# Autodesk Inventor assembly: Transmission Pulley
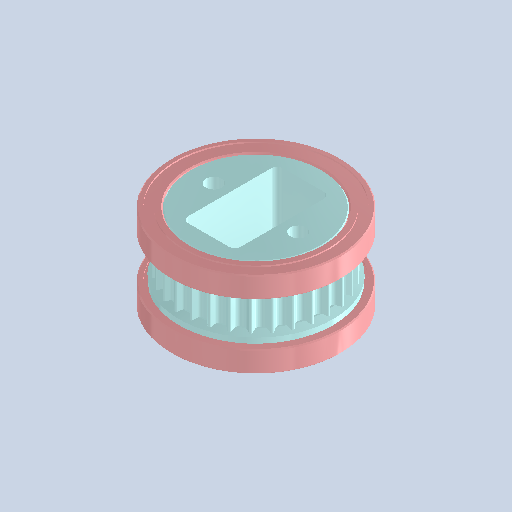
[picture p0: Inventor's stored thumbnail of the model, 512x512]
Saved by Autodesk Inventor 2023 (Build 270158000, 158)
## iProperties
Created: 2022-01-01
Part Number: Transmission Pulley
Document SubType Name: Assembly
Designer: Jochen
Author: Jochen
## Documents named in this file (3)
- D:\Projects\Lisbeth\CAD\Common\Transmission\Transmission Pulley.iam
- D:\Projects\Lisbeth\CAD\Common\Transmission\TransmissionPulleyOutput.ipt
- D:\Projects\Lisbeth\CAD\Common\Bearing\bearing_32_25_4_sbn_61705RS.ipt
## Components (3 placed, 2 different names)
1. TransmissionPulleyOutput — Mate:1, Mate:2, Mate:4, Mate:5
2. bearing_32_25_4_sbn_61705RS:1 — Mate:1, Mate:4
3. bearing_32_25_4_sbn_61705RS:2 — Mate:2, Mate:5
## Relationships (4: Mate 4)
- Mate:1: TransmissionPulleyOutput ↔ bearing_32_25_4_sbn_61705RS:1
- Mate:2: TransmissionPulleyOutput ↔ bearing_32_25_4_sbn_61705RS:2
- Mate:4: TransmissionPulleyOutput ↔ bearing_32_25_4_sbn_61705RS:1
- Mate:5: TransmissionPulleyOutput ↔ bearing_32_25_4_sbn_61705RS:2
